# Autodesk Inventor assembly: PDH_module
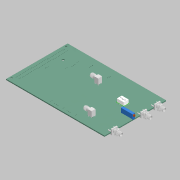
[picture p0: Inventor's stored thumbnail of the model, 180x180]
Saved by Autodesk Inventor 2021.4 (Build 254397000, 397)
## iProperties
Company: Kicad
Created: 2023-11-08
Part Number: PDH_module
Description: KiCad electronic assembly
Document SubType Name: Assembly
Designer: Tilman Preuschoff
Authority: Unknown
Sending System: KiCad to STEP converter
Preprocessor: Open CASCADE STEP processor 7.7
Title: PDH_module.step
Author: Pcbnew
## Documents named in this file (6)
- C:\Users\Tilman Preuschoff\Documents\GitHub\PDH-module\frontpanel\assembly\PDH_module.iam
- C:\Users\Tilman Preuschoff\Documents\GitHub\PDH-module\frontpanel\assembly\132289.iam
- C:\Users\Tilman Preuschoff\Documents\GitHub\PDH-module\frontpanel\assembly\901-143-3.iam
- C:\Users\Tilman Preuschoff\Documents\GitHub\PDH-module\frontpanel\assembly\User Library-SYPD-1.iam
- C:\Users\Tilman Preuschoff\Documents\GitHub\PDH-module\frontpanel\assembly\PDH_module PCB.ipt
- C:\Users\Tilman Preuschoff\Documents\GitHub\PDH-module\frontpanel\assembly\Potentiometer_Bourns_3005_Horizontal.ipt
## Components (8 placed, 8 different names)
1. 2 [sub-assembly]
2. 4 [sub-assembly]
3. 5 [sub-assembly]
4. 6 [sub-assembly]
5. 8 [sub-assembly]
6. 9 [sub-assembly]
7. 10 — Passend:1, Fluchtend:1, Tangential:1
8. Potentiometer_Bourns_3005_Horizontal:1 — Passend:1, Fluchtend:1, Tangential:1
## Relationships (3: Mate 1, Flush 1, Tangent 1)
- Passend:1 [Mate] (-0.5 mm): 10 ↔ Potentiometer_Bourns_3005_Horizontal:1
- Fluchtend:1 [Flush]: 10 ↔ Potentiometer_Bourns_3005_Horizontal:1
- Tangential:1 (-0.7 mm): 10 ↔ Potentiometer_Bourns_3005_Horizontal:1
